# Autodesk Inventor assembly: Assembly2
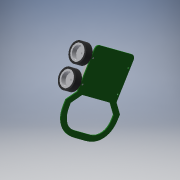
[picture p0: Inventor's stored thumbnail of the model, 180x180]
Saved by Autodesk Inventor 2016 (Build 200138000, 138)
## iProperties
Created: 2017-05-26
Part Number: Assembly2
Material: Ogólny
Document SubType Name: Assembly
Designer: Karol
Author: Karol
## Documents named in this file (7)
- D:\Git\MicromouseDixi\hardware\models\Dixi.iam
- D:\Git\MicromouseDixi\hardware\models\wheel.ipt
- D:\Git\MicromouseDixi\hardware\models\togh.ipt
- D:\Git\MicromouseDixi\hardware\models\bolt.ipt
- D:\Git\MicromouseDixi\hardware\models\tyre.ipt
- D:\Git\MicromouseDixi\hardware\models\magnet.ipt
- D:\Git\MicromouseDixi\hardware\models\mainpcb.ipt
## Components (9 placed, 6 different names)
1. mainpcb:1 — Rigid:38
2. bolt:3 — Rotational:1
3. bolt:4 — Rotational:19
4. wheel:3
5. wheel:4
6. magnet:4
7. togh:2 — Rotational:19, Rotational:1, Rigid:38
8. tyre:3
9. tyre:4
## Relationships (8: WeldJoint 6, RevoluteJoint 2)
- [WeldJoint]: bolt:4 ↔ wheel:4
- [WeldJoint]: bolt:3 ↔ wheel:3
- [WeldJoint]: bolt:4 ↔ magnet:4
- Rotational:19 [RevoluteJoint]: bolt:4 ↔ togh:2
- [WeldJoint]: wheel:3 ↔ tyre:3
- [WeldJoint]: wheel:4 ↔ tyre:4
- Rotational:1 [RevoluteJoint]: bolt:3 ↔ togh:2
- Rigid:38 [WeldJoint]: mainpcb:1 ↔ togh:2
## Named parameters: d102_d99 = 0 mm, d105_d68 = 0 mm, d106_d67 = 0 mm, d107_d21 = -4.793458 deg, d108_d22 = -0.02503 mm, d111_d4 = 0 mm, d112_d5 = 0.127925 deg, d113_d6 = 0 mm, d114_d7 = -6.839272 deg, d117_d14 = 0 mm, d118_d15 = 2.56641 deg
